# Autodesk Inventor assembly: encoder
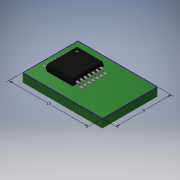
[picture p0: Inventor's stored thumbnail of the model, 180x180]
Saved by Autodesk Inventor 2018 (Build 220112000, 112)
## iProperties
Created: 2018-05-26
Part Number: encoder
Material: Ogólny
Document SubType Name: Assembly
Designer: Karol
Author: Karol
## Documents named in this file (3)
- D:\Git\MicromouseDixi\hardware\models\encoder.iam
- D:\Git\MicromouseDixi\hardware\models\tssop14.iam
- D:\Git\MicromouseDixi\hardware\models\enc_pcb.ipt
## Components (2 placed, 2 different names)
1. tssop14:1 [sub-assembly] — Zestawiający:1
2. enc_pcb:1 — Zestawiający:1
## Relationships (1: Mate 1)
- Zestawiający:1 [Mate]: tssop14:1 ↔ enc_pcb:1
